# Autodesk Inventor assembly: Front Lead Screw Idler 2
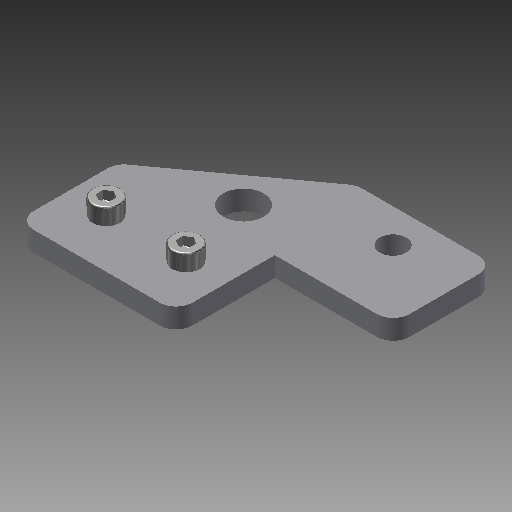
[picture p0: Inventor's stored thumbnail of the model, 512x512]
Saved by Autodesk Inventor 2018 (Build 220112000, 112)
## iProperties
Created: 2016-08-02
Part Number: Front Lead Screw Idler 2
Document SubType Name: Assembly
Designer: User
Author: User
## Documents named in this file (5)
- C:\Users\dan\OneDrive\SL-Inventor\The Beast v1.2 PackandGo\Workspaces\Workspace\Front Lead Screw Idler 2.iam
- C:\Users\dan\OneDrive\SL-Inventor\The Beast v1.2 PackandGo\Workspaces\Workspace\M5 Tee Nut-Generic_MIR.ipt
- C:\Users\dan\OneDrive\SL-Inventor\The Beast v1.2 PackandGo\Workspaces\Workspace\Leadscrew-rod-holder_MIR_MIR.ipt
- C:\Users\dan\OneDrive\SL-Inventor\The Beast v1.2 PackandGo\Workspaces\Workspace\en-US\ANSI B18.3.1M(6)\ANSI B18.3.1M - M5x0.8 x 12(1).ipt
- C:\Users\dan\OneDrive\SL-Inventor\The Beast v1.2 PackandGo\Workspaces\Workspace\M5 Tee Nut-Generic_MIR_CPY_MIR_MIR.ipt
## Components (5 placed, 4 different names)
1. M5 Tee Nut-Generic_MIR:1
2. Leadscrew-rod-holder_MIR_MIR:1
3. Forged Socket Head Cap Screw - Metric M5x0.8 x 12:1
4. Forged Socket Head Cap Screw - Metric M5x0.8 x 12:2
5. M5 Tee Nut-Generic_MIR_CPY_MIR_MIR:1
## Relationships (5: Mate 5)
- [Mate]: Leadscrew-rod-holder_MIR_MIR:1 ↔ Forged Socket Head Cap Screw - Metric M5x0.8 x 12:1
- [Mate]: Leadscrew-rod-holder_MIR_MIR:1 ↔ Forged Socket Head Cap Screw - Metric M5x0.8 x 12:1
- [Mate]: Leadscrew-rod-holder_MIR_MIR:1 ↔ Forged Socket Head Cap Screw - Metric M5x0.8 x 12:2
- [Mate]: Leadscrew-rod-holder_MIR_MIR:1 ↔ Forged Socket Head Cap Screw - Metric M5x0.8 x 12:2
- [Mate]: Forged Socket Head Cap Screw - Metric M5x0.8 x 12:2 ↔ M5 Tee Nut-Generic_MIR_CPY_MIR_MIR:1
